# Autodesk Inventor assembly: arduinomega
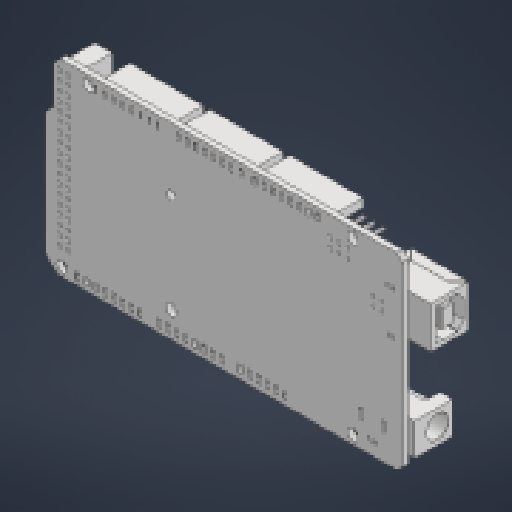
[picture p0: Inventor's stored thumbnail of the model, 512x512]
Saved by Autodesk Inventor 2026.1 (Build 301233020, 233B)
## iProperties
Created: 2025-11-26
Part Number: arduinomega
Document SubType Name: Assembly
Designer: jaewook
Author: jaewook
## Documents named in this file (3)
- C:\Users\kjh19\Documents\Inventor\project\turrte_projict_v2\arduinomega.iam
- C:\Users\kjh19\Documents\Inventor\project\turrte_projict_v2\ArduinoMega_STEP_AP203.ipt
- C:\Users\kjh19\Documents\Inventor\project\turrte_projict_v2\mega_base.ipt
## Components (2 placed, 2 different names)
1. ArduinoMega_STEP_AP203:1 — 플러쉬:1, 플러쉬:2
2. mega_base:1 — 플러쉬:1, 플러쉬:2
## Relationships (2: Flush 2)
- 플러쉬:1 [Flush]: ArduinoMega_STEP_AP203:1 ↔ mega_base:1
- 플러쉬:2 [Flush]: ArduinoMega_STEP_AP203:1 ↔ mega_base:1
